# Autodesk Inventor assembly: Assembly1
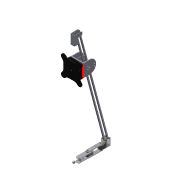
[picture p0: Inventor's stored thumbnail of the model, 180x180]
Saved by Autodesk Inventor 2011 SP1 (Build 150282100, 282)
## iProperties
Created: 2012-10-15
Part Number: Assembly1
Document SubType Name: Assembly
Designer: JohnHenry
Mass: 215.328 g
Surface Area: 1206.82 cm^2
Volume: 215.328 cm^3
Density: 1 g/cm^3
Author: JohnHenry
## Documents named in this file (28)
- C:\Users\arihon\Dropbox\Inventor\walkPivot\Assembly1.iam
- C:\Users\arihon\Dropbox\Inventor\walkPivot\JointB0.ipt
- C:\Users\arihon\Dropbox\Inventor\walkPivot\JointB1.ipt
- C:\Users\arihon\Dropbox\Inventor\walkPivot\80F-5020.ipt
- C:\Users\arihon\Dropbox\Inventor\walkPivot\JointB2.ipt
- C:\Users\arihon\Dropbox\Inventor\walkPivot\JointA2.ipt
- C:\Users\arihon\Dropbox\Inventor\walkPivot\JointA1.ipt
- C:\Users\arihon\Dropbox\Inventor\walkPivot\JointA0.ipt
- C:\Users\arihon\Dropbox\Inventor\walkPivot\JointA3.ipt
- C:\Users\arihon\Dropbox\Inventor\walkPivot\JointC0.ipt
- C:\Users\arihon\Dropbox\Inventor\walkPivot\JointC1.ipt
- C:\Users\arihon\Dropbox\Inventor\walkPivot\walkingCDGA\SLIPRING_SRG-1-6G.iam
- C:\Users\arihon\Dropbox\Inventor\walkPivot\ベアリング(仮).ipt
- C:\Users\arihon\Dropbox\Inventor\walkPivot\shaftB.ipt
- C:\Users\arihon\Dropbox\Inventor\walkPivot\JointC3.ipt
- C:\Users\arihon\Dropbox\Inventor\walkPivot\shaftC.ipt
- C:\Users\arihon\Dropbox\Inventor\walkPivot\RS30x_BottomShaft.ipt
- C:\Users\arihon\Dropbox\Inventor\walkPivot\RS30x_ServoHorn.ipt
- C:\Users\arihon\Dropbox\Inventor\walkPivot\RS30x_FreeHorn.ipt
- C:\Users\arihon\Dropbox\Inventor\walkPivot\JointC4.ipt
- C:\Users\arihon\Dropbox\Inventor\walkPivot\JointC2_.ipt
- C:\Users\arihon\Dropbox\Inventor\walkPivot\JointD1.ipt
- C:\Users\arihon\Dropbox\Inventor\walkPivot\JointD2.ipt
- C:\Users\arihon\Dropbox\Inventor\walkPivot\CounterWeight.ipt
- C:\Users\arihon\Dropbox\Inventor\walkPivot\M3_10.ipt
- C:\Users\arihon\Dropbox\Inventor\walkPivot\shaftA.ipt
- C:\Users\arihon\Dropbox\Inventor\walkPivot\JointB0_.ipt
- RS30x_FreeHorn.stp
## Components (58 placed, 26 different names)
1. JointB1:1 — メイト:1, フラッシュ:7, メイト:2, フラッシュ:19, フラッシュ:21, フラッシュ:22, 挿入:7, 挿入:8, 挿入:37, 挿入:38, 挿入:39, 挿入:40
2. JointB1:2 — フラッシュ:18, フラッシュ:20, フラッシュ:23, 挿入:6, 挿入:9, 挿入:33, 挿入:34, 挿入:35, 挿入:36
3. 80F-5020:1 — 挿入:2, 挿入:5, 挿入:43
4. JointB2:1 — メイト:1, フラッシュ:7, メイト:2
5. JointA2:1 — 挿入:2, フラッシュ:8, フラッシュ:9, フラッシュ:10, フラッシュ:12, フラッシュ:13, フラッシュ:14, フラッシュ:15, 角度:7
6. JointA1:1 — フラッシュ:8, フラッシュ:9, 挿入:3, 挿入:4, フラッシュ:11, フラッシュ:16, フラッシュ:17, メイト:7, メイト:8
7. JointA0:1 — 挿入:3, 挿入:4, メイト:6, 挿入:41, 挿入:42
8. JointA3:1 — フラッシュ:10, フラッシュ:11, フラッシュ:14, フラッシュ:17
9. JointA3:2 — フラッシュ:12, フラッシュ:13, フラッシュ:15, フラッシュ:16
10. JointB0:1 — 挿入:5, フラッシュ:18, フラッシュ:19, フラッシュ:20, フラッシュ:21, フラッシュ:22, フラッシュ:23, 角度:7, メイト:42
11. JointC1:1 — メイト:11, メイト:12, フラッシュ:27, メイト:14, メイト:16, メイト:37, メイト:41, 角度:8
12. SLIPRING_SRG-1-6G:1 [sub-assembly] — メイト:6, メイト:7, メイト:8
13. JointC0:1 — 挿入:7, 挿入:8, 挿入:12, 挿入:13, 角度:8
14. JointC0:2 — 挿入:6, 挿入:9, 挿入:10, 挿入:11
15. ベアリング(仮):1 — 挿入:13
16. ベアリング(仮):2 — 挿入:12
17. ベアリング(仮):3 — 挿入:10, メイト:9, フラッシュ:26, メイト:12
18. ベアリング(仮):4 — 挿入:11, メイト:10, フラッシュ:25
19. shaftB:1 — メイト:10, フラッシュ:25, メイト:13
20. shaftB:2 — メイト:9, フラッシュ:26, メイト:11
21. JointC1:2 — メイト:13, フラッシュ:27, メイト:15, メイト:38
22. JointC3:1 — 挿入:14, 挿入:15, 挿入:16, 挿入:17, フラッシュ:28, フラッシュ:29, メイト:25, メイト:26, メイト:27, 角度:6
23. ベアリング(仮):5 — 挿入:17, メイト:18
24. ベアリング(仮):6 — 挿入:14
25. ベアリング(仮):7 — 挿入:15, メイト:14, メイト:16
26. ベアリング(仮):8 — 挿入:16, メイト:15, メイト:17
27. shaftC:1 — メイト:18, フラッシュ:29
28. shaftC:2 — メイト:17, フラッシュ:28
29. RS30x_BottomShaft:1 — メイト:21, メイト:22, メイト:23, フラッシュ:31, フラッシュ:32, メイト:25, メイト:26, メイト:27
30. RS30x_BottomShaft:2 — メイト:19, メイト:20, メイト:24, フラッシュ:30, フラッシュ:32, 角度:5, メイト:31, メイト:32, メイト:33, メイト:34, メイト:35, メイト:36
31. RS30x_ServoHorn:1 — メイト:21, メイト:22, 挿入:18, 挿入:19
32. RS30x_ServoHorn:2 — メイト:19, メイト:20, 挿入:22, 挿入:23
33. RS30x_FreeHorn:1 — メイト:24, フラッシュ:30, 挿入:27, 挿入:28
34. RS30x_FreeHorn:2 — メイト:23, フラッシュ:31, 挿入:20, 挿入:21
35. JointC4:1 — 挿入:18, 挿入:19, 挿入:22, 挿入:23, 角度:5, 角度:6
36. JointC4:2 — 挿入:20, 挿入:21, 挿入:27, 挿入:28
37. JointC2_:1 — メイト:31, メイト:32, メイト:33, 挿入:24, 挿入:25
38. JointC2_:2 — メイト:34, メイト:35, メイト:36
39. JointD1:1 — 挿入:24, 挿入:25, 挿入:26
40. JointD2:1 — 挿入:26
41. CounterWeight:1 — 挿入:29, 挿入:30, 挿入:31, 挿入:32, メイト:41
42. ベアリング(仮):9 — 挿入:30
43. ベアリング(仮):10 — 挿入:31, メイト:39
44. ベアリング(仮):11 — 挿入:32, フラッシュ:34
45. ベアリング(仮):12 — 挿入:29, メイト:40, フラッシュ:33
46. shaftC:3 — メイト:38, メイト:39, フラッシュ:34
47. shaftC:4 — メイト:37, メイト:40, フラッシュ:33
48. M3_10:1 — 挿入:33
49. M3_10:2 — 挿入:36
50. M3_10:3 — 挿入:35
51. M3_10:4 — 挿入:34
52. M3_10:5 — 挿入:37
53. M3_10:6 — 挿入:38
54. M3_10:7 — 挿入:40
55. M3_10:8 — 挿入:39
56. shaftA:1 — 挿入:41
57. ベアリング(仮):13 — 挿入:42
58. JointB0_:1 — メイト:42, 挿入:43
## Relationships (109: Insert 42, Mate 36, Flush 27, Angle 4)
- メイト:1 [Mate] (0.1 mm): JointB1:1 ↔ JointB2:1
- フラッシュ:7 [Flush]: JointB1:1 ↔ JointB2:1
- メイト:2 [Mate]: JointB1:1 ↔ JointB2:1
- 挿入:2 [Insert]: 80F-5020:1 ↔ JointA2:1
- フラッシュ:8 [Flush]: JointA2:1 ↔ JointA1:1
- フラッシュ:9 [Flush]: JointA2:1 ↔ JointA1:1
- 挿入:3 [Insert]: JointA1:1 ↔ JointA0:1
- 挿入:4 [Insert]: JointA1:1 ↔ JointA0:1
- フラッシュ:10 [Flush]: JointA2:1 ↔ JointA3:1
- フラッシュ:11 [Flush]: JointA1:1 ↔ JointA3:1
- フラッシュ:12 [Flush]: JointA2:1 ↔ JointA3:2
- フラッシュ:13 [Flush]: JointA2:1 ↔ JointA3:2
- フラッシュ:14 [Flush]: JointA2:1 ↔ JointA3:1
- フラッシュ:15 [Flush]: JointA2:1 ↔ JointA3:2
- フラッシュ:16 [Flush]: JointA1:1 ↔ JointA3:2
- フラッシュ:17 [Flush]: JointA1:1 ↔ JointA3:1
- 挿入:5 [Insert]: 80F-5020:1 ↔ JointB0:1
- フラッシュ:18 [Flush]: JointB1:2 ↔ JointB0:1
- フラッシュ:19 [Flush]: JointB1:1 ↔ JointB0:1
- フラッシュ:20 [Flush]: JointB1:2 ↔ JointB0:1
- フラッシュ:21 [Flush]: JointB1:1 ↔ JointB0:1
- フラッシュ:22 [Flush]: JointB1:1 ↔ JointB0:1
- フラッシュ:23 [Flush]: JointB1:2 ↔ JointB0:1
- メイト:6 [Mate]: JointA0:1 ↔ SLIPRING_SRG-1-6G:1
- メイト:7 [Mate]: JointA1:1 ↔ SLIPRING_SRG-1-6G:1
- メイト:8 [Mate]: JointA1:1 ↔ SLIPRING_SRG-1-6G:1
- 挿入:6 [Insert]: JointB1:2 ↔ JointC0:2
- 挿入:7 [Insert]: JointB1:1 ↔ JointC0:1
- 挿入:8 [Insert]: JointB1:1 ↔ JointC0:1
- 挿入:9 [Insert]: JointB1:2 ↔ JointC0:2
- 挿入:10 [Insert]: JointC0:2 ↔ ベアリング(仮):3
- 挿入:11 [Insert]: JointC0:2 ↔ ベアリング(仮):4
- 挿入:12 [Insert]: JointC0:1 ↔ ベアリング(仮):2
- 挿入:13 [Insert]: JointC0:1 ↔ ベアリング(仮):1
- メイト:9 [Mate]: ベアリング(仮):3 ↔ shaftB:2
- メイト:10 [Mate]: ベアリング(仮):4 ↔ shaftB:1
- フラッシュ:25 [Flush] (3 mm): ベアリング(仮):4 ↔ shaftB:1
- フラッシュ:26 [Flush] (3 mm): ベアリング(仮):3 ↔ shaftB:2
- メイト:11 [Mate]: JointC1:1 ↔ shaftB:2
- メイト:12 [Mate] (9.5 mm): JointC1:1 ↔ ベアリング(仮):3
- メイト:13 [Mate]: shaftB:1 ↔ JointC1:2
- フラッシュ:27 [Flush]: JointC1:1 ↔ JointC1:2
- 挿入:14 [Insert]: JointC3:1 ↔ ベアリング(仮):6
- 挿入:15 [Insert]: JointC3:1 ↔ ベアリング(仮):7
- 挿入:16 [Insert]: JointC3:1 ↔ ベアリング(仮):8
- 挿入:17 [Insert]: JointC3:1 ↔ ベアリング(仮):5
- メイト:14 [Mate]: JointC1:1 ↔ ベアリング(仮):7
- メイト:15 [Mate]: JointC1:2 ↔ ベアリング(仮):8
- メイト:16 [Mate] (10 mm): JointC1:1 ↔ ベアリング(仮):7
- メイト:17 [Mate]: ベアリング(仮):8 ↔ shaftC:2
- メイト:18 [Mate]: ベアリング(仮):5 ↔ shaftC:1
- フラッシュ:28 [Flush]: JointC3:1 ↔ shaftC:2
- フラッシュ:29 [Flush]: JointC3:1 ↔ shaftC:1
- メイト:19 [Mate]: RS30x_BottomShaft:2 ↔ RS30x_ServoHorn:2
- メイト:20 [Mate]: RS30x_BottomShaft:2 ↔ RS30x_ServoHorn:2
- メイト:21 [Mate]: RS30x_BottomShaft:1 ↔ RS30x_ServoHorn:1
- メイト:22 [Mate]: RS30x_BottomShaft:1 ↔ RS30x_ServoHorn:1
- メイト:23 [Mate]: RS30x_BottomShaft:1 ↔ RS30x_FreeHorn:2
- メイト:24 [Mate]: RS30x_BottomShaft:2 ↔ RS30x_FreeHorn:1
- フラッシュ:30 [Flush]: RS30x_BottomShaft:2 ↔ RS30x_FreeHorn:1
- フラッシュ:31 [Flush]: RS30x_BottomShaft:1 ↔ RS30x_FreeHorn:2
- フラッシュ:32 [Flush]: RS30x_BottomShaft:1 ↔ RS30x_BottomShaft:2
- メイト:25 [Mate]: JointC3:1 ↔ RS30x_BottomShaft:1
- メイト:26 [Mate]: JointC3:1 ↔ RS30x_BottomShaft:1
- メイト:27 [Mate]: JointC3:1 ↔ RS30x_BottomShaft:1
- 挿入:18 [Insert]: RS30x_ServoHorn:1 ↔ JointC4:1
- 挿入:19 [Insert]: RS30x_ServoHorn:1 ↔ JointC4:1
- 挿入:20 [Insert]: RS30x_FreeHorn:2 ↔ JointC4:2
- 挿入:21 [Insert]: RS30x_FreeHorn:2 ↔ JointC4:2
- 挿入:22 [Insert]: RS30x_ServoHorn:2 ↔ JointC4:1
- 挿入:23 [Insert]: RS30x_ServoHorn:2 ↔ JointC4:1
- 角度:5 [Angle] (0 deg): RS30x_BottomShaft:2 ↔ JointC4:1
- メイト:31 [Mate]: RS30x_BottomShaft:2 ↔ JointC2_:1
- メイト:32 [Mate]: RS30x_BottomShaft:2 ↔ JointC2_:1
- メイト:33 [Mate]: RS30x_BottomShaft:2 ↔ JointC2_:1
- メイト:34 [Mate]: RS30x_BottomShaft:2 ↔ JointC2_:2
- メイト:35 [Mate]: RS30x_BottomShaft:2 ↔ JointC2_:2
- メイト:36 [Mate]: RS30x_BottomShaft:2 ↔ JointC2_:2
- 挿入:24 [Insert] (0.1 mm): JointC2_:1 ↔ JointD1:1
- 挿入:25 [Insert] (0.1 mm): JointC2_:1 ↔ JointD1:1
- 挿入:26 [Insert]: JointD1:1 ↔ JointD2:1
- 挿入:27 [Insert]: RS30x_FreeHorn:1 ↔ JointC4:2
- 挿入:28 [Insert]: RS30x_FreeHorn:1 ↔ JointC4:2
- 角度:6 [Angle] (0 deg): JointC3:1 ↔ JointC4:1
- 挿入:29 [Insert]: CounterWeight:1 ↔ ベアリング(仮):12
- 挿入:30 [Insert]: CounterWeight:1 ↔ ベアリング(仮):9
- 挿入:31 [Insert]: CounterWeight:1 ↔ ベアリング(仮):10
- 挿入:32 [Insert]: CounterWeight:1 ↔ ベアリング(仮):11
- メイト:37 [Mate]: JointC1:1 ↔ shaftC:4
- メイト:38 [Mate]: JointC1:2 ↔ shaftC:3
- メイト:39 [Mate]: ベアリング(仮):10 ↔ shaftC:3
- メイト:40 [Mate]: ベアリング(仮):12 ↔ shaftC:4
- フラッシュ:33 [Flush]: ベアリング(仮):12 ↔ shaftC:4
- フラッシュ:34 [Flush]: ベアリング(仮):11 ↔ shaftC:3
- メイト:41 [Mate] (10.5 mm): JointC1:1 ↔ CounterWeight:1
- 角度:7 [Angle] (0 deg): JointA2:1 ↔ JointB0:1
- 角度:8 [Angle] (15 deg): JointC1:1 ↔ JointC0:1
- 挿入:33 [Insert]: JointB1:2 ↔ M3_10:1
- 挿入:34 [Insert]: JointB1:2 ↔ M3_10:4
- 挿入:35 [Insert]: JointB1:2 ↔ M3_10:3
- 挿入:36 [Insert]: JointB1:2 ↔ M3_10:2
- 挿入:37 [Insert]: JointB1:1 ↔ M3_10:5
- 挿入:38 [Insert]: JointB1:1 ↔ M3_10:6
- 挿入:39 [Insert]: JointB1:1 ↔ M3_10:8
- 挿入:40 [Insert]: JointB1:1 ↔ M3_10:7
- 挿入:41 [Insert]: JointA0:1 ↔ shaftA:1
- 挿入:42 [Insert] (0.5 mm): JointA0:1 ↔ ベアリング(仮):13
- メイト:42 [Mate]: JointB0:1 ↔ JointB0_:1
- 挿入:43 [Insert] (0.1 mm): 80F-5020:1 ↔ JointB0_:1
